# Autodesk Inventor assembly: 22-128Z2-PHTM-HRDSET
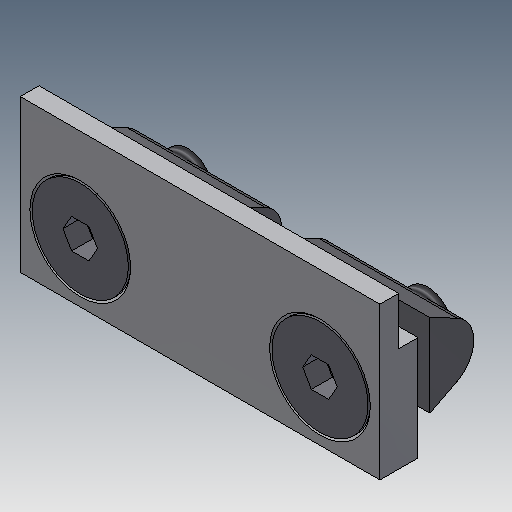
[picture p0: Inventor's stored thumbnail of the model, 512x512]
Saved by Autodesk Inventor 2018.3 (Build 223284000, 284)
## iProperties
Created: 2004-11-24
Part Number: 22-128Z2-PHTM-HRDSET
Document SubType Name: Assembly
Designer: Autodesk, Inc.
Manufacturer: Standard
Standards Organization: Custom
Mass: 58.1662 g
Surface Area: 79.3674 cm^2
Volume: 11.8873 cm^3
Density: 4.89315 g/cm^3
CAGE: 1LJX3
Dept. ID: Product Design
Description #2: ---
Finish #1: ---
Finish #2: ---
Material ID: ---
Project Number: ---
Author: Autodesk, Inc.
## Documents named in this file (6)
- C:\AVAInvAPI\Workspace\Test Station\Components\22-128Z2 Hardware Set.iam
- C:\AVAInvAPI\Workspace\Test Station\Components\22-128Z2.ipt
- C:\AVAInvAPI\Workspace\Test Station\Components\24-218-8.ipt
- C:\AVAInvAPI\Workspace\Test Station\Components\20-058.ipt
- C:\Users\kelleyb.ADS\Desktop\Samples MIGRATED 2009 224 RTM_1\Standard Parts\Test Station Content\Fastners\2X-YYY-ZZ IPS Screws.ipt
- C:\Users\kelleyb.ADS\Desktop\Samples MIGRATED 2009 224 RTM_1\Standard Parts\Test Station Content\Fastners\20-XXX TSlot Nuts.ipt
## Components (5 placed, 3 different names)
1. 22-128Z2:1 — Insert:1, Mate:2, Angle:1, Insert:2, Angle:2
2. 24-218-8:1 — Insert:1, Mate:1
3. 20-058:1 — Mate:1, Mate:2, Angle:1, Flush:1
4. 24-218-8:3 — Insert:2, Mate:3
5. 20-058:2 — Mate:3, Flush:1, Angle:2
## Relationships (8: Mate 3, Insert 2, Angle 2, Flush 1)
- Insert:1: 22-128Z2:1 ↔ 24-218-8:1
- Mate:1: 24-218-8:1 ↔ 20-058:1
- Mate:2 (4.5 mm): 22-128Z2:1 ↔ 20-058:1
- Angle:1 (-90 deg): 22-128Z2:1 ↔ 20-058:1
- Insert:2: 22-128Z2:1 ↔ 24-218-8:3
- Mate:3: 24-218-8:3 ↔ 20-058:2
- Flush:1: 20-058:1 ↔ 20-058:2
- Angle:2 (0 deg): 22-128Z2:1 ↔ 20-058:2
